# Autodesk Inventor assembly: !towers
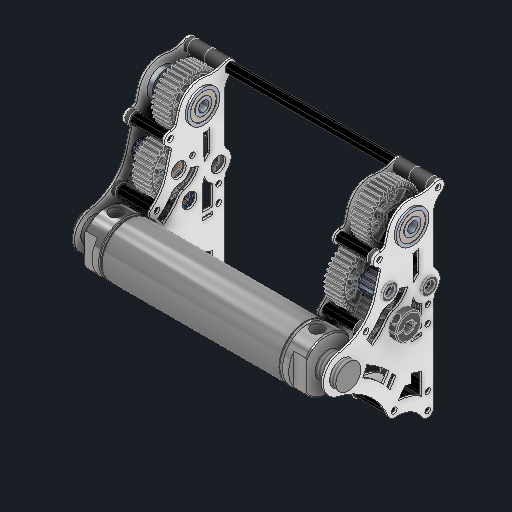
[picture p0: Inventor's stored thumbnail of the model, 512x512]
Saved by Autodesk Inventor 2024 (Build 280153000, 153)
## iProperties
Created: 2023-11-21
Part Number: !towers
Document SubType Name: Assembly
Designer: avere
Author: avere
## Documents named in this file (7)
- C:\Users\avere\Documents\rbp_cad\zoomba_v0.1\arm\!towers.iam
- C:\Users\avere\Documents\rbp_cad\zoomba_v0.1\arm\gearbox.iam
- gearbox.iam
- C:\Users\avere\Documents\rbp_cad\zoomba_v0.1\arm\mirrored_parts\gearbox_MIR.iam
- C:\Users\avere\Documents\rbp_cad\VEX-CAD-Inventor-1.41\Structure\Standoff\Standoff 5.00.ipt
- C:\Users\avere\Documents\rbp_cad\VEX-CAD-Inventor-1.41\Structure\Standoff.ipt
- C:\Users\avere\Documents\rbp_cad\VEX-CAD-Inventor-1.41\Motion\Pneumatics\Reservoir.ipt
## Components (4 placed, 4 different names)
1. gearbox:1 [sub-assembly] — Insert:1, Insert:3, Mate:1
2. gearbox_MIR:1 [sub-assembly] — Insert:1, Insert:2, Mate:1
3. Standoff 5.00:1 — Insert:2
4. Reservoir:1 — Insert:3
## Relationships (4: Insert 3, Mate 1)
- Insert:1 (127 mm): gearbox:1 ↔ gearbox_MIR:1
- Insert:2: gearbox_MIR:1 ↔ Standoff 5.00:1
- Insert:3 (-4.7625 mm): gearbox:1 ↔ Reservoir:1
- Mate:1: gearbox:1 ↔ gearbox_MIR:1
